# Autodesk Inventor assembly: prototype v2
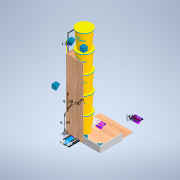
[picture p0: Inventor's stored thumbnail of the model, 180x180]
Saved by Autodesk Inventor 2020 (Build 240168000, 168)
## iProperties
Created: 2021-02-27
Part Number: prototype v2
Document SubType Name: Assembly
Designer: Bernard Li
Author: Bernard Li
## Documents named in this file (11)
- C:\Users\Johnl\Documents\Li Industries\AngelCAD\prototype v2.iam
- C:\Users\Johnl\Documents\Li Industries\AngelCAD\panel connector.ipt
- C:\Users\Johnl\Documents\Li Industries\AngelCAD\Shared Files\17g servo.ipt
- C:\Users\Johnl\Documents\Li Industries\AngelCAD\cup noodle.ipt
- C:\Users\Johnl\Documents\Li Industries\AngelCAD\grounplate.ipt
- C:\Users\Johnl\Documents\Li Industries\AngelCAD\side panel 1.ipt
- C:\Users\Johnl\Documents\Li Industries\AngelCAD\moving plate.ipt
- C:\Users\Johnl\Documents\Li Industries\AngelCAD\support paneling.ipt
- C:\Users\Johnl\Documents\Li Industries\AngelCAD\cover2.ipt
- C:\Users\Johnl\Documents\Li Industries\AngelCAD\motor mount v2.ipt
- C:\Users\Johnl\Documents\Li Industries\AngelCAD\Shared Files\arduino uno.ipt
## Components (23 placed, 10 different names)
1. grounplate:1 — Mate:1, Mate:2, Mate:5, Mate:6, Mate:8, Mate:9, Flush:3, Flush:4, Mate:30, Mate:32, Mate:39, Mate:40, Mate:45
2. panel connector:1 — Mate:1, Mate:6, Flush:3, Flush:5, Mate:11, Mate:31
3. panel connector:3 — Mate:2, Mate:8, Flush:4, Mate:22
4. panel connector:4 — Mate:5, Mate:9, Mate:28, Mate:29
5. side panel 1:1 — Flush:5, Mate:11, Flush:8, Mate:24, Mate:25, Mate:26, Mate:27, Flush:9, Mate:28, Mate:29, Tangent:1, Flush:11, Flush:13
6. moving plate:1 — Mate:16, Mate:17
7. panel connector:5 — Mate:24, Mate:25, Flush:13
8. support paneling:1 — Mate:31, Flush:10, Flush:11, Mate:33, Flush:12, Mate:34
9. cover2:1 — Mate:22, Flush:8, Flush:10
10. panel connector:6 — Mate:26, Mate:27, Flush:9
11. panel connector:7 — Mate:32
12. panel connector:8 — Mate:33, Flush:12, Mate:34
13. panel connector:9
14. motor mount v2:1 — Mate:35, Mate:36, Mate:37
15. motor mount v2:2 — Mate:39, Mate:40, Mate:42, Mate:43, Mate:44, Mate:45
16. arduino uno:1
17. cup noodle:1 — Mate:30, Tangent:1
18. cup noodle:2
19. cup noodle:3
20. cup noodle:4
21. cup noodle:5
22. 17g servo:1 — Mate:16, Mate:17, Mate:42, Mate:43, Mate:44
23. 17g servo:2 — Mate:35, Mate:36, Mate:37
## Relationships (40: Mate 30, Flush 9, Tangent 1)
- Mate:1: grounplate:1 ↔ panel connector:1
- Mate:2: grounplate:1 ↔ panel connector:3
- Mate:5: grounplate:1 ↔ panel connector:4
- Mate:6: grounplate:1 ↔ panel connector:1
- Mate:8: grounplate:1 ↔ panel connector:3
- Mate:9: grounplate:1 ↔ panel connector:4
- Flush:3: grounplate:1 ↔ panel connector:1
- Flush:4: grounplate:1 ↔ panel connector:3
- Flush:5: panel connector:1 ↔ side panel 1:1
- Mate:11: panel connector:1 ↔ side panel 1:1
- Mate:16: moving plate:1 ↔ 17g servo:1
- Mate:17: moving plate:1 ↔ 17g servo:1
- Mate:22: panel connector:3 ↔ cover2:1
- Flush:8: side panel 1:1 ↔ cover2:1
- Mate:24: side panel 1:1 ↔ panel connector:5
- Mate:25: side panel 1:1 ↔ panel connector:5
- Mate:26: side panel 1:1 ↔ panel connector:6
- Mate:27 (3.175 mm): side panel 1:1 ↔ panel connector:6
- Flush:9: side panel 1:1 ↔ panel connector:6
- Mate:28: panel connector:4 ↔ side panel 1:1
- Mate:29: panel connector:4 ↔ side panel 1:1
- Mate:30: grounplate:1 ↔ cup noodle:1
- Tangent:1: side panel 1:1 ↔ cup noodle:1
- Mate:31: panel connector:1 ↔ support paneling:1
- Flush:10: support paneling:1 ↔ cover2:1
- Flush:11: side panel 1:1 ↔ support paneling:1
- Mate:32: grounplate:1 ↔ panel connector:7
- Mate:33: support paneling:1 ↔ panel connector:8
- Flush:12: support paneling:1 ↔ panel connector:8
- Mate:34 (3.429 mm): support paneling:1 ↔ panel connector:8
- Flush:13: side panel 1:1 ↔ panel connector:5
- Mate:35: motor mount v2:1 ↔ 17g servo:2
- Mate:36: motor mount v2:1 ↔ 17g servo:2
- Mate:37: motor mount v2:1 ↔ 17g servo:2
- Mate:39: grounplate:1 ↔ motor mount v2:2
- Mate:40: grounplate:1 ↔ motor mount v2:2
- Mate:42: motor mount v2:2 ↔ 17g servo:1
- Mate:43: motor mount v2:2 ↔ 17g servo:1
- Mate:44: motor mount v2:2 ↔ 17g servo:1
- Mate:45 (20 mm): grounplate:1 ↔ motor mount v2:2
